# Autodesk Inventor assembly: ASY ДМФ 030 кольцо со шпильками корма v2.0
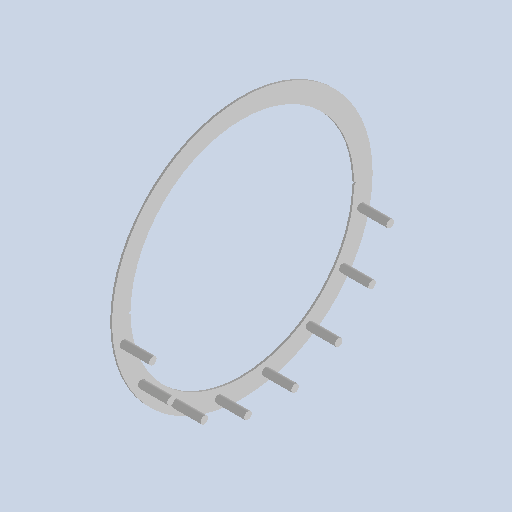
[picture p0: Inventor's stored thumbnail of the model, 512x512]
Saved by Autodesk Inventor 2025 (Build 290162010, 162A)
## iProperties
Created: 2024-04-23
Part Number: ASY ДМФ 030 кольцо со шпильками корма v2.0
Document SubType Name: Assembly
Designer: admin
Author: admin
## Documents named in this file (4)
- C:\Users\pokla\Documents\Inventor\ДФО\ДМФ\DMF-Disk-Micro-Filter\ASY ДМФ 030 кольцо со шпильками корма v2.0.iam
- C:\Users\pokla\Documents\Inventor\ДФО\ДМФ\DMF-Disk-Micro-Filter\ДМФ 031 кольцо под шпильки НОС v2.0.ipt
- C:\Users\pokla\Documents\Inventor\ДФО\ДМФ\DMF-Disk-Micro-Filter\ДМФ 000 размеры v2.0.ipt
- C:\Users\pokla\Documents\Inventor\ДФО\ДМФ\DMF-Disk-Micro-Filter\ДМС 033 шпилька 3 v2.0.ipt
## Components (9 placed, 2 different names)
1. ДМФ 031 кольцо под шпильки НОС v2.0.ipt:1 — Mate:1, Rigid:1
2. ДМС 033 шпилька 3 v2.0.ipt:1 — Rigid:1
3. ДМС 033 шпилька 3 v2.0.ipt:2
4. ДМС 033 шпилька 3 v2.0.ipt:3
5. ДМС 033 шпилька 3 v2.0.ipt:4
6. ДМС 033 шпилька 3 v2.0.ipt:5
7. ДМС 033 шпилька 3 v2.0.ipt:6
8. ДМС 033 шпилька 3 v2.0.ipt:7
9. ДМС 033 шпилька 3 v2.0.ipt:8
## Component patterns: (8 elements, first: ДМС 033 шпилька 3 v2.0.ipt:1)
## Relationships (2: Mate 1, WeldJoint 1)
- Mate:1: ДМФ 031 кольцо под шпильки НОС v2.0.ipt:1
- Rigid:1 [WeldJoint]: ДМФ 031 кольцо под шпильки НОС v2.0.ipt:1 ↔ ДМС 033 шпилька 3 v2.0.ipt:1
